# Autodesk Inventor assembly: Сборка1
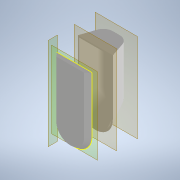
[picture p0: Inventor's stored thumbnail of the model, 180x180]
Saved by Autodesk Inventor 2022.1 (Build 261234000, 234)
## iProperties
Created: 2021-12-14
Part Number: Сборка1
Document SubType Name: Assembly
Designer: Grigori
Author: Grigori
## Documents named in this file (3)
- C:\Users\Grigo\Desktop\Дрон\Сборка\Сборка1.iam
- C:\Users\Grigo\Desktop\Дрон\Сборка\Корпус.ipt
- C:\Users\Grigo\Desktop\Дрон\Сборка\Крышка корпуса.ipt
## Components (2 placed, 2 different names)
1. Корпус:1 — Жесткий:1, Жесткий:2
2. Крышка корпуса:1 — Жесткий:1, Жесткий:2
## Relationships (2: WeldJoint 2)
- Жесткий:1 [WeldJoint]: Корпус:1 ↔ Крышка корпуса:1
- Жесткий:2 [WeldJoint]: Корпус:1 ↔ Крышка корпуса:1
